# Autodesk Inventor assembly: 3A.03.JS.Wing test assembly_CPY
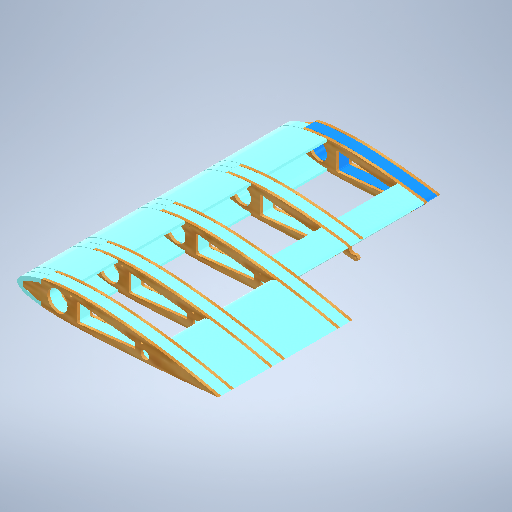
[picture p0: Inventor's stored thumbnail of the model, 512x512]
Saved by Autodesk Inventor 2025.1 (Build 291241000, 241)
## iProperties
Created: 2025-01-14
Part Number: 3A.03.JS.Wing test assembly_CPY
Document SubType Name: Assembly
Designer: johan
Author: johan
## Documents named in this file (14)
- C:\Users\johan\OneDrive - University of Bristol\CAD docs\2) Wing\Avionics Cradle\3A.03.01.JS.Wing test assembly Avoinics Cradle.iam
- C:\Users\johan\OneDrive - University of Bristol\CAD docs\2) Wing\2) Ribs\assemblies\3A.01.09.JS.Rib 9_CPY.iam
- C:\Users\johan\OneDrive - University of Bristol\CAD docs\2) Wing\2) Ribs\assemblies\3A.01.10.JS.Rib 10_CPY.iam
- C:\Users\johan\OneDrive - University of Bristol\CAD docs\2) Wing\2) Ribs\assemblies\3A.01.11.JS.Rib 11_CPY.iam
- C:\Users\johan\OneDrive - University of Bristol\CAD docs\2) Wing\2) Ribs\assemblies\3A.01.12.JS.Rib 12_CPY.iam
- C:\Users\johan\OneDrive - University of Bristol\CAD docs\2) Wing\2) Ribs\assemblies\3A.01.13.JS.Rib 13_CPY.iam
- C:\Users\johan\OneDrive - University of Bristol\CAD docs\2) Wing\3) Leading edge\assemblies\3A.04.01.JS.54mm root_CPY.iam
- C:\Users\johan\OneDrive - University of Bristol\CAD docs\2) Wing\3) Leading edge\assemblies\3A.04.02.JS.77mm_CPY.iam
- C:\Users\johan\OneDrive - University of Bristol\CAD docs\2) Wing\3) Leading edge\assemblies\3A.04.03.JS.74.75mm_CPY.iam
- C:\Users\johan\OneDrive - University of Bristol\CAD docs\2) Wing\3) Leading edge\assemblies\3A.04.04.90.75mm_CPY.iam
- C:\Users\johan\OneDrive - University of Bristol\CAD docs\2) Wing\4) Trailing edge\3P.05.07.JS.flap trailing edge 90_CPY.ipt
- C:\Users\johan\OneDrive - University of Bristol\CAD docs\2) Wing\4) Trailing edge\3P.05.01.JS.trailing edge 54mm_CPY.ipt
- C:\Users\johan\OneDrive - University of Bristol\CAD docs\2) Wing\4) Trailing edge\3P.05.06.JS.flap trailing edge 74_CPY.ipt
- C:\Users\johan\OneDrive - University of Bristol\CAD docs\2) Wing\4) Trailing edge\3P.05.02.JS.trailing edge 77mm_CPY.ipt
## Components (13 placed, 13 different names)
1. 3A.01.09.JS.Rib 9_CPY:1 [sub-assembly] — Rigid:8
2. 3A.01.10.JS.Rib 10_CPY:1 [sub-assembly] — Rigid:6, Rigid:7, Rigid:25, Rigid:30
3. 3A.01.11.JS.Rib 11_CPY:1 [sub-assembly] — Rigid:4, Rigid:5
4. 3A.01.12.JS.Rib 12_CPY:1 [sub-assembly] — Rigid:2, Rigid:3, Rigid:39
5. 3A.01.13.JS.Rib 13_CPY:1 [sub-assembly] — Rigid:27, Rigid:26
6. 3A.04.01.JS.54mm root_CPY:1 [sub-assembly] — Rigid:27, Rigid:2
7. 3A.04.02.JS.77mm_CPY:1 [sub-assembly] — Rigid:4, Rigid:3
8. 3A.04.03.JS.74.75mm_CPY:1 [sub-assembly] — Rigid:6, Rigid:5
9. 3A.04.04.90.75mm_CPY:1 [sub-assembly] — Rigid:8, Rigid:7
10. 3P.05.07.JS.flap trailing edge 90_CPY:1 — Rigid:25
11. 3P.05.01.JS.trailing edge 54mm_CPY:1 — Rigid:26
12. 3P.05.06.JS.flap trailing edge 74_CPY:1 — Rigid:30
13. 3P.05.02.JS.trailing edge 77mm_CPY:1 — Rigid:39
## Relationships (12: WeldJoint 12)
- Rigid:27 [WeldJoint]: 3A.01.13.JS.Rib 13_CPY:1 ↔ 3A.04.01.JS.54mm root_CPY:1
- Rigid:2 [WeldJoint]: 3A.01.12.JS.Rib 12_CPY:1 ↔ 3A.04.01.JS.54mm root_CPY:1
- Rigid:4 [WeldJoint]: 3A.01.11.JS.Rib 11_CPY:1 ↔ 3A.04.02.JS.77mm_CPY:1
- Rigid:3 [WeldJoint]: 3A.01.12.JS.Rib 12_CPY:1 ↔ 3A.04.02.JS.77mm_CPY:1
- Rigid:6 [WeldJoint]: 3A.01.10.JS.Rib 10_CPY:1 ↔ 3A.04.03.JS.74.75mm_CPY:1
- Rigid:5 [WeldJoint]: 3A.01.11.JS.Rib 11_CPY:1 ↔ 3A.04.03.JS.74.75mm_CPY:1
- Rigid:8 [WeldJoint]: 3A.01.09.JS.Rib 9_CPY:1 ↔ 3A.04.04.90.75mm_CPY:1
- Rigid:7 [WeldJoint]: 3A.01.10.JS.Rib 10_CPY:1 ↔ 3A.04.04.90.75mm_CPY:1
- Rigid:25 [WeldJoint]: 3A.01.10.JS.Rib 10_CPY:1 ↔ 3P.05.07.JS.flap trailing edge 90_CPY:1
- Rigid:26 [WeldJoint]: 3A.01.13.JS.Rib 13_CPY:1 ↔ 3P.05.01.JS.trailing edge 54mm_CPY:1
- Rigid:30 [WeldJoint]: 3A.01.10.JS.Rib 10_CPY:1 ↔ 3P.05.06.JS.flap trailing edge 74_CPY:1
- Rigid:39 [WeldJoint]: 3A.01.12.JS.Rib 12_CPY:1 ↔ 3P.05.02.JS.trailing edge 77mm_CPY:1
